# Autodesk Inventor assembly: Head
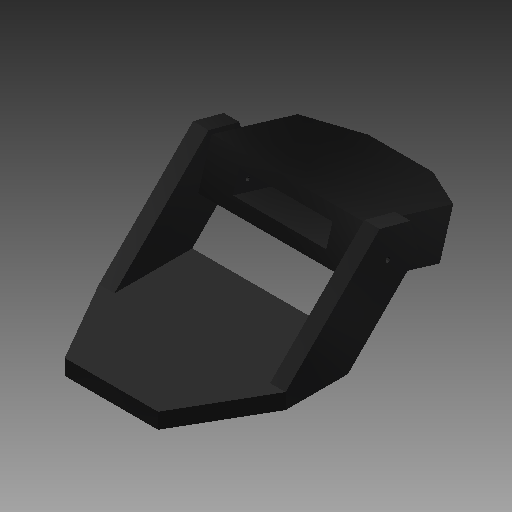
[picture p0: Inventor's stored thumbnail of the model, 512x512]
Saved by Autodesk Inventor 2017 (Build 210142000, 142)
## iProperties
Created: 2018-10-18
Part Number: Head
Document SubType Name: Assembly
Designer: Dell
Author: Dell
## Documents named in this file (4)
- C:\Users\Dell\Documents\GitHub\tr2\Head\Head.iam
- C:\Users\Dell\Documents\GitHub\tr2\Head\HA01.ipt
- C:\Users\Dell\Documents\GitHub\tr2\Head\Orbbec Astra\Orbbec Astra.iam
- C:\Users\Dell\Documents\GitHub\tr2\Head\HA02.ipt
## Components (3 placed, 3 different names)
1. HA01:1 — Mate:1, Flush:1, Mate:2, Mate:7
2. Orbbec Astra:1 [sub-assembly] — Mate:1, Flush:1
3. HA02:1 — Mate:2, Mate:4, Mate:5, Mate:6, Mate:7
## Relationships (7: Mate 6, Flush 1)
- Mate:1 (2 mm): HA01:1 ↔ Orbbec Astra:1
- Flush:1 (-20 mm): HA01:1 ↔ Orbbec Astra:1
- Mate:2: HA01:1 ↔ HA02:1
- Mate:4: HA02:1
- Mate:5 (125 mm): HA02:1
- Mate:6: HA02:1
- Mate:7: HA01:1 ↔ HA02:1
